# Autodesk Inventor assembly: AXb3
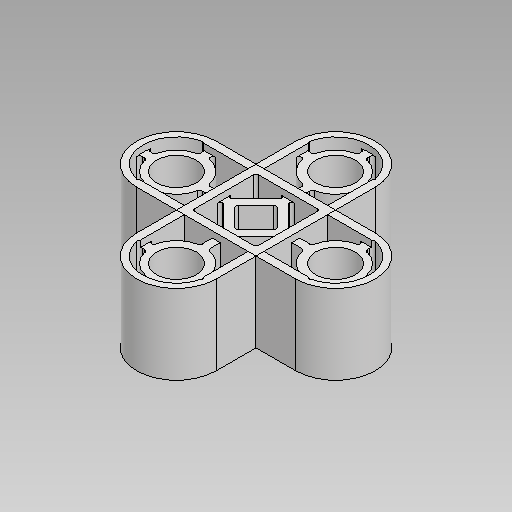
[picture p0: Inventor's stored thumbnail of the model, 512x512]
Saved by Autodesk Inventor 2020 (Build 240168000, 168)
## iProperties
Created: 2019-05-06
Part Number: AXb3
Document SubType Name: Assembly
Designer: Varga Daniel
Author: Varga Daniel
## Documents named in this file (3)
- C:\!_Dani\!_cloud\OneDrive\!_munka\Revolution\StructuralParts\Beams\Axle Beams\AXb3.iam
- C:\!_Dani\!_cloud\OneDrive\!_munka\Revolution\StructuralParts\Beams\Axle Beams\Axle beam base.ipt
- C:\!_Dani\!_cloud\OneDrive\!_munka\Revolution\StructuralParts\Beams\beam_single_end_part.ipt
## Components (5 placed, 2 different names)
1. Axle beam base:1 — Mate:1, Mate:2, Flush:1, Mate:3, Mate:4, Mate:5, Mate:6, Flush:2, Flush:3, Flush:4, Flush:5, Flush:6, Flush:7, Flush:8, Flush:9
2. beam_single_end_part:1 — Mate:4, Flush:2, Flush:9
3. beam_single_end_part:2 — Mate:5, Flush:3, Flush:8
4. beam_single_end_part:3 — Mate:6, Flush:5, Flush:6
5. beam_single_end_part:4 — Mate:3, Flush:4, Flush:7
## Relationships (15: Flush 9, Mate 6)
- Mate:1: Axle beam base:1
- Mate:2: Axle beam base:1
- Flush:1: Axle beam base:1
- Mate:3: Axle beam base:1 ↔ beam_single_end_part:4
- Mate:4: Axle beam base:1 ↔ beam_single_end_part:1
- Mate:5: Axle beam base:1 ↔ beam_single_end_part:2
- Mate:6: Axle beam base:1 ↔ beam_single_end_part:3
- Flush:2: Axle beam base:1 ↔ beam_single_end_part:1
- Flush:3: Axle beam base:1 ↔ beam_single_end_part:2
- Flush:4: Axle beam base:1 ↔ beam_single_end_part:4
- Flush:5: Axle beam base:1 ↔ beam_single_end_part:3
- Flush:6: Axle beam base:1 ↔ beam_single_end_part:3
- Flush:7: Axle beam base:1 ↔ beam_single_end_part:4
- Flush:8: Axle beam base:1 ↔ beam_single_end_part:2
- Flush:9: Axle beam base:1 ↔ beam_single_end_part:1
